# Autodesk Inventor assembly: t-slot_mount_2inx1in_assembly
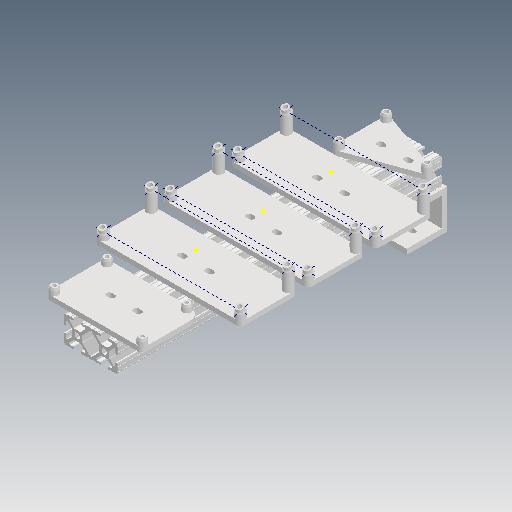
[picture p0: Inventor's stored thumbnail of the model, 512x512]
Saved by Autodesk Inventor 2025.1 (Build 291241000, 241)
## iProperties
Created: 2026-07-04
Part Number: t-slot_mount_2inx1in_assembly
Document SubType Name: Assembly
Designer: Aiden
Author: Aiden
## Documents named in this file (6)
- C:\Users\Aiden\Documents\GitHub\coldex-instrumentation\hardware\mounting_hardware\t-slot_mount_2inx1inx12in\t-slot_mount_2inx1in_assembly.iam
- C:\Users\Aiden\Documents\GitHub\coldex-instrumentation\hardware\mounting_hardware\t-slot_mount_2inx1inx12in\47065T418_T-Slotted Framing.ipt
- C:\Users\Aiden\Documents\GitHub\coldex-instrumentation\hardware\mounting_hardware\t-slot_mount_2inx1inx12in\db-25_standoffs_plate_t-slot-2inx1in.ipt
- C:\Users\Aiden\Documents\GitHub\coldex-instrumentation\hardware\mounting_hardware\t-slot_mount_2inx1inx12in\relay_module_standoffs_angled_plate_t-slot-2inx1in.ipt
- C:\Users\Aiden\Documents\GitHub\coldex-instrumentation\hardware\mounting_hardware\t-slot_mount_2inx1inx12in\arduino_mega_standoffs_plate_t-slot-2inx1in.ipt
- C:\Users\Aiden\Documents\GitHub\coldex-instrumentation\hardware\mounting_hardware\t-slot_mount_2inx1inx12in\hanging_bracket_t-slot-2inx1in.ipt
## Components (7 placed, 5 different names)
1. 47065T418_T-Slotted Framing:1 — Mate:1, Mate:2, Mate:3, Mate:4
2. db-25_standoffs_plate_t-slot-2inx1in:1 — Mate:1
3. arduino_mega_standoffs_plate_t-slot-2inx1in:1 — Mate:3
4. hanging_bracket_t-slot-2inx1in:1 — Mate:4
5. relay_module_standoffs_angled_plate_t-slot-2inx1in:1 — Mate:2
6. relay_module_standoffs_angled_plate_t-slot-2inx1in:2
7. relay_module_standoffs_angled_plate_t-slot-2inx1in:3
## Component patterns: (3 elements, first: relay_module_standoffs_angled_plate_t-slot-2inx1in:1)
## Relationships (4: Mate 4)
- Mate:1: 47065T418_T-Slotted Framing:1 ↔ db-25_standoffs_plate_t-slot-2inx1in:1
- Mate:2: 47065T418_T-Slotted Framing:1 ↔ relay_module_standoffs_angled_plate_t-slot-2inx1in:1
- Mate:3: 47065T418_T-Slotted Framing:1 ↔ arduino_mega_standoffs_plate_t-slot-2inx1in:1
- Mate:4: 47065T418_T-Slotted Framing:1 ↔ hanging_bracket_t-slot-2inx1in:1
